# Autodesk Inventor assembly: Drive
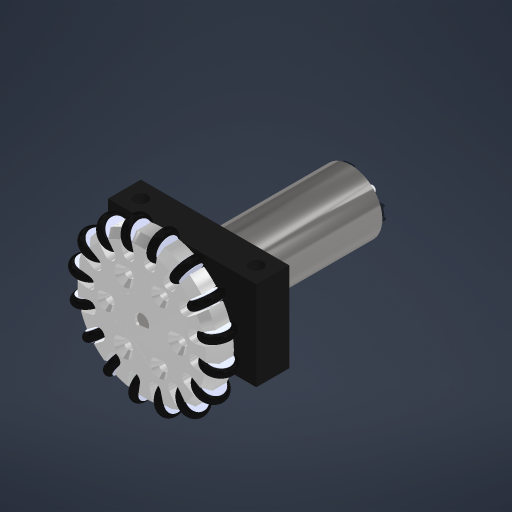
[picture p0: Inventor's stored thumbnail of the model, 512x512]
Saved by Autodesk Inventor 2023 (Build 270158000, 158)
## iProperties
Created: 2023-05-12
Part Number: Drive
Document SubType Name: Assembly
Designer: Elias Braun
Author: Elias Braun
## Documents named in this file (4)
- C:\Users\Elias Braun\Nextcloud2\RoboCup2023\Motor\Drive.iam
- C:\Users\Elias Braun\Nextcloud2\RoboCup2023\Motor\MotorBracket.ipt
- C:\Users\Elias Braun\Nextcloud2\RoboCup2023\Motor\Maxon\B7B9384D898D.iam
- C:\Users\Elias Braun\Nextcloud2\RoboCup2023\Motor\Wheel\Rad.iam
## Components (3 placed, 3 different names)
1. MotorBracket:1 — Mate:1, Mate:2, Mate:3, Mate:5
2. B7B9384D898D:1 [sub-assembly] — Mate:1, Mate:2, Mate:3, Mate:4
3. Rad:1 [sub-assembly] — Mate:4, Mate:5
## Relationships (5: Mate 5)
- Mate:1: MotorBracket:1 ↔ B7B9384D898D:1
- Mate:2: MotorBracket:1 ↔ B7B9384D898D:1
- Mate:3: MotorBracket:1 ↔ B7B9384D898D:1
- Mate:4: B7B9384D898D:1 ↔ Rad:1
- Mate:5: MotorBracket:1 ↔ Rad:1
